# Autodesk Inventor assembly: RobotAndLowBar
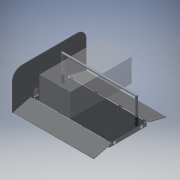
[picture p0: Inventor's stored thumbnail of the model, 180x180]
Saved by Autodesk Inventor 2016 SP1 (Build 200210100, 210)
## iProperties
Created: 2016-01-17
Part Number: RobotAndLowBar
Document SubType Name: Assembly
Designer: steele
Author: steele
## Documents named in this file (3)
- C:\snobotics\CAD-Development\robSteele\SnoBotics2016\RobotAndLowBar.iam
- C:\snobotics\CAD-Development\robSteele\SnoBotics2016\FieldElements\rdsLowBar.iam
- C:\snobotics\CAD-Development\robSteele\SnoBotics2016\VolumeShapes\catapultMaxVolume.ipt
## Components (2 placed, 2 different names)
1. rdsLowBar:1 [sub-assembly] — Mate:1, Mate:2, Flush:1
2. catapultMaxVolume:1 — Mate:1, Mate:2, Flush:1
## Relationships (3: Mate 2, Flush 1)
- Mate:1: rdsLowBar:1 ↔ catapultMaxVolume:1
- Mate:2 (127 mm): rdsLowBar:1 ↔ catapultMaxVolume:1
- Flush:1: rdsLowBar:1 ↔ catapultMaxVolume:1
